# Autodesk Inventor assembly: HyperCube Evolution - Double Z motor 1.0
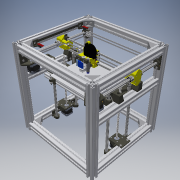
[picture p0: Inventor's stored thumbnail of the model, 180x180]
Saved by Autodesk Inventor 2016 (Build 200138000, 138)
## iProperties
Created: 2017-04-14
Part Number: HyperCube Evolution - Double Z motor 1.0
Document SubType Name: Assembly
Designer: Scott
Author: Scott
## Documents named in this file (18)
- E:\Scott Projects\3D Printing\CoreXY\HyperCube Evolution - Double Z motor 1.0.iam
- E:\Scott Projects\3D Printing\CoreXY\HyperCube Evolution.iam
- E:\Scott Projects\3D Printing\CoreXY\3030 Extrusion - Y.ipt
- E:\Scott Projects\3D Printing\CoreXY\Z Axis Liner Rail Bracket Assembly - Left 1.0.iam
- E:\Scott Projects\3D Printing\CoreXY\Z Axis Liner Rail Bracket Assembly - Right 1.0.iam
- E:\Scott Projects\3D Printing\CoreXY\X Axis Assembly 1.0.iam
- E:\Scott Projects\3D Printing\CoreXY\X Carriage Assembly.iam
- E:\Scott Projects\3D Printing\CoreXY\Extruder Assembly.iam
- E:\Scott Projects\3D Printing\CoreXY\Linear rail - Double Z.ipt
- E:\Scott Projects\3D Printing\CoreXY\Build Platform Assembly - Double Z - 1.0.iam
- E:\Scott Projects\3D Printing\CoreXY\Z Axis Liner Rail Bracket Assembly - Tall - Left 1.0.iam
- E:\Scott Projects\3D Printing\CoreXY\Z Axis Liner Rail Bracket Assembly - Tall - Right 1.0.iam
- E:\Scott Projects\3D Printing\CoreXY\Z Motor Mount Assembly 1.0.iam
- E:\Scott Projects\3D Printing\CoreXY\Y End Stop Assembly.iam
- E:\Scott Projects\3D Printing\CoreXY\T Slot Cover 250mm.ipt
- E:\Scott Projects\3D Printing\CoreXY\GT2_20T.ipt
- E:\Scott Projects\3D Printing\CoreXY\Belt 3.ipt
- E:\Scott Projects\3D Printing\CoreXY\Belt 4.ipt
## Components (29 placed, 17 different names)
1. HyperCube Evolution:1 [sub-assembly] — Flush:1, Flush:2, Flush:3, Mate:1, Flush:4, Flush:5, Mate:2, Flush:6, Mate:3, Mate:4, Mate:5, Mate:6, Mate:7, Mate:8, Mate:9, Mate:10, Mate:11, Mate:12, Mate:49, Mate:50, Mate:52, Mate:53, Flush:10, Mate:55, Mate:56, Flush:11, Mate:57, Mate:58, Mate:59, Mate:60, Mate:61, Mate:62, Mate:64, Mate:65, Mate:66, Mate:67, Mate:75, Mate:76
2. 3030 Extrusion - Y:1 — Mate:1, Flush:4, Flush:5, Flush:7, Mate:38, Mate:39, Mate:45, Mate:46
3. 3030 Extrusion - Y:2 — Mate:2, Flush:6, Flush:7, Mate:37, Mate:40, Mate:43, Mate:44
4. Z Axis Liner Rail Bracket Assembly - Left 1.0:1 [sub-assembly] — Mate:3, Mate:4, Insert:1
5. Z Axis Liner Rail Bracket Assembly - Left 1.0:2 [sub-assembly] — Mate:5, Mate:6, Insert:3
6. Z Axis Liner Rail Bracket Assembly - Right 1.0:1 [sub-assembly] — Mate:7, Mate:10, Insert:4
7. Z Axis Liner Rail Bracket Assembly - Right 1.0:2 [sub-assembly] — Mate:8, Mate:9, Insert:2
8. X Axis Assembly 1.0:1 [sub-assembly] — Mate:11, Mate:12, Mate:13, Mate:14, Flush:14, Flush:15, Mate:69, Mate:70, Mate:77, Mate:79, Mate:82
9. X Carriage Assembly:1 [sub-assembly] — Mate:13, Mate:14, Flush:8, Mate:15, Flush:9, Mate:71, Mate:72, Mate:78, Mate:80
10. Extruder Assembly:1 [sub-assembly] — Flush:8, Mate:15, Flush:9, Mate:82
11. Linear rail - Double Z:1 — Insert:2, Mate:19, Mate:41
12. Linear rail - Double Z:2 — Insert:1, Mate:18, Mate:48
13. Linear rail - Double Z:3 — Insert:3, Mate:17, Mate:47
14. Linear rail - Double Z:4 — Insert:4, Mate:16, Mate:42
15. Build Platform Assembly - Double Z - 1.0:1 [sub-assembly] — Mate:16, Mate:17, Mate:18, Mate:19, Mate:51, Mate:54, Flush:10
16. Z Axis Liner Rail Bracket Assembly - Tall - Left 1.0:1 [sub-assembly] — Mate:38, Mate:39, Mate:42
17. Z Axis Liner Rail Bracket Assembly - Tall - Left 1.0:2 [sub-assembly] — Mate:37, Mate:40, Mate:41
18. Z Axis Liner Rail Bracket Assembly - Tall - Right 1.0:1 [sub-assembly] — Mate:43, Mate:44, Mate:48
19. Z Axis Liner Rail Bracket Assembly - Tall - Right 1.0:2 [sub-assembly] — Mate:45, Mate:46, Mate:47
20. Z Motor Mount Assembly 1.0:1 [sub-assembly] — Mate:49, Mate:50, Mate:51
21. Z Motor Mount Assembly 1.0:2 [sub-assembly] — Mate:52, Mate:53, Mate:54
22. Y End Stop Assembly:1 [sub-assembly] — Mate:57, Mate:58, Flush:12
23. Y End Stop Assembly:2 [sub-assembly] — Mate:55, Mate:56, Flush:11, Flush:12
24. T Slot Cover 250mm:1 — Mate:59, Mate:60, Mate:63
25. T Slot Cover 250mm:2 — Mate:61, Mate:62, Flush:13
26. GT2_20T:1 — Mate:65, Flush:14, Mate:74, Mate:81
27. GT2_20T:2 — Mate:64, Flush:15, Mate:68, Mate:73
28. Belt 3:1 — Mate:66, Mate:67, Mate:68, Mate:69, Mate:70, Mate:71, Mate:72, Mate:73
29. Belt 4:1 — Mate:74, Mate:75, Mate:76, Mate:77, Mate:78, Mate:79, Mate:80, Mate:81
## Relationships (84: Mate 65, Flush 15, Insert 4)
- Flush:1: HyperCube Evolution:1
- Flush:2: HyperCube Evolution:1
- Flush:3: HyperCube Evolution:1
- Mate:1: HyperCube Evolution:1 ↔ 3030 Extrusion - Y:1
- Flush:4: HyperCube Evolution:1 ↔ 3030 Extrusion - Y:1
- Flush:5 (130 mm): HyperCube Evolution:1 ↔ 3030 Extrusion - Y:1
- Mate:2: HyperCube Evolution:1 ↔ 3030 Extrusion - Y:2
- Flush:6: HyperCube Evolution:1 ↔ 3030 Extrusion - Y:2
- Flush:7: 3030 Extrusion - Y:1 ↔ 3030 Extrusion - Y:2
- Mate:3: HyperCube Evolution:1 ↔ Z Axis Liner Rail Bracket Assembly - Left 1.0:1
- Mate:4: HyperCube Evolution:1 ↔ Z Axis Liner Rail Bracket Assembly - Left 1.0:1
- Mate:5: HyperCube Evolution:1 ↔ Z Axis Liner Rail Bracket Assembly - Left 1.0:2
- Mate:6: HyperCube Evolution:1 ↔ Z Axis Liner Rail Bracket Assembly - Left 1.0:2
- Mate:7: HyperCube Evolution:1 ↔ Z Axis Liner Rail Bracket Assembly - Right 1.0:1
- Mate:8: HyperCube Evolution:1 ↔ Z Axis Liner Rail Bracket Assembly - Right 1.0:2
- Mate:9: HyperCube Evolution:1 ↔ Z Axis Liner Rail Bracket Assembly - Right 1.0:2
- Mate:10: HyperCube Evolution:1 ↔ Z Axis Liner Rail Bracket Assembly - Right 1.0:1
- Mate:11: HyperCube Evolution:1 ↔ X Axis Assembly 1.0:1
- Mate:12: HyperCube Evolution:1 ↔ X Axis Assembly 1.0:1
- Mate:13: X Axis Assembly 1.0:1 ↔ X Carriage Assembly:1
- Mate:14: X Axis Assembly 1.0:1 ↔ X Carriage Assembly:1
- Flush:8: X Carriage Assembly:1 ↔ Extruder Assembly:1
- Mate:15: X Carriage Assembly:1 ↔ Extruder Assembly:1
- Flush:9: X Carriage Assembly:1 ↔ Extruder Assembly:1
- Insert:1: Z Axis Liner Rail Bracket Assembly - Left 1.0:1 ↔ Linear rail - Double Z:2
- Insert:2: Z Axis Liner Rail Bracket Assembly - Right 1.0:2 ↔ Linear rail - Double Z:1
- Insert:3: Z Axis Liner Rail Bracket Assembly - Left 1.0:2 ↔ Linear rail - Double Z:3
- Insert:4: Z Axis Liner Rail Bracket Assembly - Right 1.0:1 ↔ Linear rail - Double Z:4
- Mate:16: Linear rail - Double Z:4 ↔ Build Platform Assembly - Double Z - 1.0:1
- Mate:17: Linear rail - Double Z:3 ↔ Build Platform Assembly - Double Z - 1.0:1
- Mate:18: Linear rail - Double Z:2 ↔ Build Platform Assembly - Double Z - 1.0:1
- Mate:19: Linear rail - Double Z:1 ↔ Build Platform Assembly - Double Z - 1.0:1
- Mate:37: 3030 Extrusion - Y:2 ↔ Z Axis Liner Rail Bracket Assembly - Tall - Left 1.0:2
- Mate:38: 3030 Extrusion - Y:1 ↔ Z Axis Liner Rail Bracket Assembly - Tall - Left 1.0:1
- Mate:39: 3030 Extrusion - Y:1 ↔ Z Axis Liner Rail Bracket Assembly - Tall - Left 1.0:1
- Mate:40: 3030 Extrusion - Y:2 ↔ Z Axis Liner Rail Bracket Assembly - Tall - Left 1.0:2
- Mate:41: Linear rail - Double Z:1 ↔ Z Axis Liner Rail Bracket Assembly - Tall - Left 1.0:2
- Mate:42: Linear rail - Double Z:4 ↔ Z Axis Liner Rail Bracket Assembly - Tall - Left 1.0:1
- Mate:43: 3030 Extrusion - Y:2 ↔ Z Axis Liner Rail Bracket Assembly - Tall - Right 1.0:1
- Mate:44: 3030 Extrusion - Y:2 ↔ Z Axis Liner Rail Bracket Assembly - Tall - Right 1.0:1
- Mate:45: 3030 Extrusion - Y:1 ↔ Z Axis Liner Rail Bracket Assembly - Tall - Right 1.0:2
- Mate:46: 3030 Extrusion - Y:1 ↔ Z Axis Liner Rail Bracket Assembly - Tall - Right 1.0:2
- Mate:47: Linear rail - Double Z:3 ↔ Z Axis Liner Rail Bracket Assembly - Tall - Right 1.0:2
- Mate:48: Linear rail - Double Z:2 ↔ Z Axis Liner Rail Bracket Assembly - Tall - Right 1.0:1
- Mate:49: HyperCube Evolution:1 ↔ Z Motor Mount Assembly 1.0:1
- Mate:50: HyperCube Evolution:1 ↔ Z Motor Mount Assembly 1.0:1
- Mate:51: Build Platform Assembly - Double Z - 1.0:1 ↔ Z Motor Mount Assembly 1.0:1
- Mate:52: HyperCube Evolution:1 ↔ Z Motor Mount Assembly 1.0:2
- Mate:53: HyperCube Evolution:1 ↔ Z Motor Mount Assembly 1.0:2
- Mate:54: Build Platform Assembly - Double Z - 1.0:1 ↔ Z Motor Mount Assembly 1.0:2
- Flush:10: HyperCube Evolution:1 ↔ Build Platform Assembly - Double Z - 1.0:1
- Mate:55: HyperCube Evolution:1 ↔ Y End Stop Assembly:2
- Mate:56: HyperCube Evolution:1 ↔ Y End Stop Assembly:2
- Flush:11 (5 mm): HyperCube Evolution:1 ↔ Y End Stop Assembly:2
- Mate:57: HyperCube Evolution:1 ↔ Y End Stop Assembly:1
- Mate:58: HyperCube Evolution:1 ↔ Y End Stop Assembly:1
- Flush:12: Y End Stop Assembly:1 ↔ Y End Stop Assembly:2
- Mate:59: HyperCube Evolution:1 ↔ T Slot Cover 250mm:1
- Mate:60 (0.1 mm): HyperCube Evolution:1 ↔ T Slot Cover 250mm:1
- Mate:61: HyperCube Evolution:1 ↔ T Slot Cover 250mm:2
- Mate:62 (0.1 mm): HyperCube Evolution:1 ↔ T Slot Cover 250mm:2
- Flush:13: T Slot Cover 250mm:2
- Mate:63: T Slot Cover 250mm:1
- Mate:64: HyperCube Evolution:1 ↔ GT2_20T:2
- Mate:65: HyperCube Evolution:1 ↔ GT2_20T:1
- Flush:14: X Axis Assembly 1.0:1 ↔ GT2_20T:1
- Flush:15: X Axis Assembly 1.0:1 ↔ GT2_20T:2
- Mate:66: HyperCube Evolution:1 ↔ Belt 3:1
- Mate:67: HyperCube Evolution:1 ↔ Belt 3:1
- Mate:68: GT2_20T:2 ↔ Belt 3:1
- Mate:69: X Axis Assembly 1.0:1 ↔ Belt 3:1
- Mate:70: X Axis Assembly 1.0:1 ↔ Belt 3:1
- Mate:71: X Carriage Assembly:1 ↔ Belt 3:1
- Mate:72: X Carriage Assembly:1 ↔ Belt 3:1
- Mate:73 (0.25 mm): GT2_20T:2 ↔ Belt 3:1
- Mate:74: GT2_20T:1 ↔ Belt 4:1
- Mate:75: HyperCube Evolution:1 ↔ Belt 4:1
- Mate:76: HyperCube Evolution:1 ↔ Belt 4:1
- Mate:77: X Axis Assembly 1.0:1 ↔ Belt 4:1
- Mate:78: X Carriage Assembly:1 ↔ Belt 4:1
- Mate:79: X Axis Assembly 1.0:1 ↔ Belt 4:1
- Mate:80: X Carriage Assembly:1 ↔ Belt 4:1
- Mate:81 (0.25 mm): GT2_20T:1 ↔ Belt 4:1
- Mate:82 (100 mm): X Axis Assembly 1.0:1 ↔ Extruder Assembly:1
